# Autodesk Inventor assembly: Assembly5
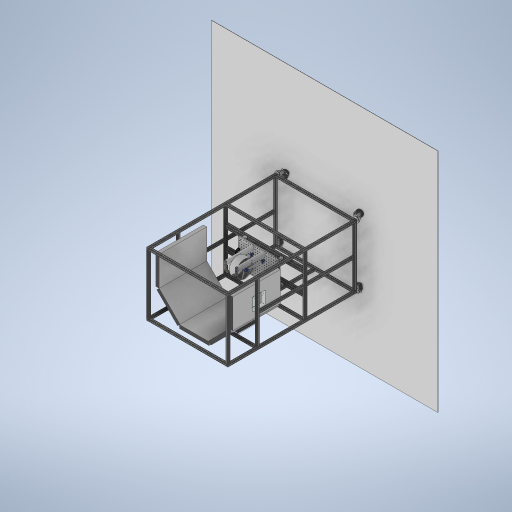
[picture p0: Inventor's stored thumbnail of the model, 512x512]
Saved by Autodesk Inventor 2024 (Build 280153000, 153)
## iProperties
Created: 2021-07-16
Part Number: Assembly5
Document SubType Name: Assembly
Designer: negre
Author: negre
## Documents named in this file (14)
- C:\Users\rosam\OneDrive\Documents\github_latest\Hardware\Tablet-Rig\Assemblies\Frame_training.iam
- C:\Users\rosam\OneDrive\Documents\github_latest\Hardware\Tablet-Rig\Parts\McMaster-Carr 47065T801\47065T801_T-Slotted Framing_57-inches.ipt
- C:\Users\rosam\OneDrive\Documents\github_latest\Hardware\Tablet-Rig\Parts\McMaster-Carr 47065T919\47065T919_T-Slotted Framing_caster.ipt
- C:\Users\rosam\OneDrive\Documents\github_latest\Hardware\Tablet-Rig\Assemblies\Wheel_w_board.iam
- C:\Users\rosam\OneDrive\Documents\github_latest\Hardware\Tablet-Rig\Parts\ThorLabs RS2\RS2-Step.ipt
- C:\Users\rosam\OneDrive\Documents\github_latest\Hardware\Tablet-Rig\Parts\McMaster-Carr 47065T801\47065T801_T-Slotted Framing_21-inches.ipt
- C:\Users\rosam\OneDrive\Documents\github_latest\Hardware\Tablet-Rig\Assemblies\Monitors_VESA-mountable.iam
- C:\Users\rosam\OneDrive\Documents\github_latest\Hardware\Tablet-Rig\Parts\Ground.ipt
- C:\Users\rosam\OneDrive\Documents\github_latest\Hardware\Tablet-Rig\Parts\McMaster-Carr 47065T801\47065T801_T-Slotted Framing_34-inches.ipt
- C:\Users\rosam\OneDrive\Documents\github_latest\Hardware\Tablet-Rig\Parts\McMaster-Carr 47065T803\47065T803_T-Slotted Framing_34-inches.ipt
- C:\Users\rosam\OneDrive\Documents\github_latest\Hardware\Tablet-Rig\Parts\McMaster-Carr 47065T801\47065T801_T-Slotted Framing_26-inches.ipt
- C:\Users\rosam\OneDrive\Documents\github_latest\Hardware\Tablet-Rig\Parts\McMaster-Carr 47065T801\47065T801_T-Slotted Framing_20-inches.ipt
- C:\Users\rosam\OneDrive\Documents\github_latest\Hardware\Tablet-Rig\Parts\VESA adapter bracket.ipt
- C:\Users\rosam\OneDrive\Documents\github_latest\Hardware\Tablet-Rig\Parts\McMaster-Carr 47065T801\47065T801_T-Slotted Framing_11-inches.ipt
## Components (46 placed, 13 different names)
1. 47065T801_T-Slotted Framing_57-inches:1 — Mate:1087, Mate:1088, Flush:895, Flush:1074, Flush:1075, Flush:1077, Flush:1079, Flush:1081, Mate:1282, Mate:1307, Flush:1144, Flush:1145, Mate:1309, Flush:1146, Flush:1155
2. 47065T801_T-Slotted Framing_57-inches:2 — Mate:1085, Mate:1086, Flush:1083, Flush:1084, Flush:1087, Mate:1281, Flush:1089, Mate:1305, Symmetry:1, Mate:1308, Mate:1311, Flush:1149, Mate:1313, Flush:1154, Flush:1193
3. 47065T801_T-Slotted Framing_57-inches:3 — Mate:1091, Mate:1092, Flush:895, Flush:1069, Mate:1275, Flush:1072, Flush:1073, Mate:1276, Flush:1076, Mate:1277, Flush:1078, Mate:1278, Flush:1080, Flush:1141, Flush:1142, Mate:1316, Flush:1160, Flush:1166, Flush:1167, Flush:1169
4. 47065T801_T-Slotted Framing_57-inches:4 — Mate:1089, Mate:1090, Mate:1279, Flush:1082, Flush:1085, Mate:1280, Flush:1086, Flush:1090, Flush:1141, Flush:1143, Symmetry:1, Mate:1321, Flush:1164, Flush:1165, Mate:1322, Flush:1168, Mate:1323, Mate:1327, Flush:1178, Mate:1330, Flush:1192
5. 47065T919_T-Slotted Framing_caster:1 — Mate:1087, Mate:1088
6. 47065T919_T-Slotted Framing_caster:2 — Mate:1091, Mate:1092
7. 47065T919_T-Slotted Framing_caster:3 — Mate:1089, Mate:1090
8. 47065T919_T-Slotted Framing_caster:4 — Mate:1085, Mate:1086, Mate:1274
9. Wheel_w_board:1 [sub-assembly] — Mate:1107, Mate:1108, Mate:1109, Mate:1110, Mate:1111, Mate:1112, Mate:1113, Mate:1114, Angle:1, Angle:2, Flush:1066, Flush:1067, Flush:1068, Flush:1136, Flush:1139
10. RS2-Step:1 — Mate:1107, Mate:1114, Mate:1302
11. RS2-Step:2 — Mate:1110, Mate:1111
12. RS2-Step:3 — Mate:1108, Mate:1113, Mate:1304
13. RS2-Step:4 — Mate:1109, Mate:1112
14. 47065T801_T-Slotted Framing_21-inches:1 — Mate:1310, Flush:1152, Mate:1312, Flush:1183, Flush:1184
15. 47065T801_T-Slotted Framing_21-inches:2 — Mate:1325, Flush:1176, Mate:1328, Flush:1182, Flush:1184
16. Monitors_VESA-mountable:1 [sub-assembly] — Angle:1, Angle:2, Flush:1066, Flush:1067, Flush:1068, Flush:1069, Angle:3, Angle:4, Flush:1071, Mate:1273, Mate:1318, Mate:1332, Flush:1186, Mate:1336, Flush:1190, Flush:1191, Flush:1194, Flush:1195, Flush:1196
17. Ground:1 — Mate:1270, Mate:1271, Flush:1070, Angle:3, Angle:4, Flush:1071, Mate:1273, Mate:1274, Angle:5, Mate:1306
18. 47065T801_T-Slotted Framing_34-inches:1 — Mate:1275, Flush:1072, Flush:1073, Flush:1074, Flush:1075, Mate:1282, Flush:1188, Flush:1189
19. 47065T801_T-Slotted Framing_34-inches:2 — Mate:1276, Flush:1076, Flush:1077, Flush:1147
20. 47065T801_T-Slotted Framing_34-inches:3 — Mate:1277, Flush:1078, Flush:1079, Flush:1091, Mate:1317, Flush:1162, Flush:1172
21. 47065T801_T-Slotted Framing_34-inches:4 — Mate:1278, Flush:1080, Flush:1081, Flush:1088, Flush:1140, Flush:1142, Flush:1151, Mate:1319, Flush:1163, Flush:1180
22. 47065T801_T-Slotted Framing_34-inches:5 — Mate:1279, Flush:1082, Flush:1083, Flush:1084, Flush:1085
23. 47065T801_T-Slotted Framing_34-inches:6 — Mate:1280, Flush:1086, Flush:1087, Flush:1088, Mate:1305, Flush:1140, Angle:5, Flush:1143, Flush:1150, Flush:1179
24. 47065T801_T-Slotted Framing_34-inches:7 — Mate:1281, Flush:1089, Flush:1090, Flush:1091, Flush:1148
25. 47065T803_T-Slotted Framing_34-inches:1 — Mate:1304, Flush:1139, Flush:1156, Flush:1174
26. 47065T803_T-Slotted Framing_34-inches:2 — Mate:1302, Flush:1136, Flush:1157, Mate:1324, Flush:1173, Mate:1326
27. 47065T801_T-Slotted Framing_26-inches:1 — Mate:1309, Flush:1146, Flush:1147, Flush:1148, Mate:1310, Flush:1152, Flush:1156, Flush:1157, Mate:1314, Flush:1158, Flush:1175, Mate:1326
28. 47065T801_T-Slotted Framing_26-inches:2 — Mate:1327, Flush:1178, Mate:1328, Flush:1179, Flush:1180
29. 47065T801_T-Slotted Framing_26-inches:3 — Mate:1323, Mate:1324, Flush:1172, Flush:1173, Flush:1174, Flush:1175, Mate:1325, Flush:1176, Mate:1329, Flush:1181
30. 47065T801_T-Slotted Framing_26-inches:4 — Mate:1322, Flush:1168, Flush:1169, Flush:1170, Flush:1171, Mate:1339
31. 47065T801_T-Slotted Framing_26-inches:5 — Mate:1307, Flush:1144, Flush:1145, Mate:1308, Flush:1185, Flush:1187
32. 47065T801_T-Slotted Framing_26-inches:6 — Mate:1311, Flush:1149, Flush:1150, Flush:1151, Mate:1312
33. 47065T801_T-Slotted Framing_26-inches:7 — Mate:1321, Flush:1164, Flush:1165, Flush:1166, Flush:1167
34. 47065T801_T-Slotted Framing_26-inches:8 — Mate:1313, Flush:1154, Flush:1155, Mate:1315, Flush:1161, Flush:1171, Mate:1331, Mate:1333
35. 47065T801_T-Slotted Framing_20-inches:1 — Mate:1314, Flush:1158, Mate:1315, Flush:1183
36. 47065T801_T-Slotted Framing_34-inches:8 — Mate:1316, Flush:1160, Flush:1161, Flush:1170, Mate:1335, Mate:1337
37. 47065T801_T-Slotted Framing_20-inches:2 — Mate:1317, Flush:1162, Mate:1318, Mate:1320
38. 47065T801_T-Slotted Framing_21-inches:3 — Mate:1319, Flush:1163, Mate:1320
39. 47065T801_T-Slotted Framing_20-inches:3 — Mate:1329, Flush:1181, Flush:1182, Mate:1330
40. VESA adapter bracket:1 — Mate:1338, Flush:1190, Flush:1194
41. VESA adapter bracket:2 — Mate:1331, Flush:1185, Flush:1193
42. VESA adapter bracket:3 — Mate:1339, Flush:1191, Flush:1192
43. VESA adapter bracket:4 — Mate:1334, Flush:1187, Flush:1196
44. VESA adapter bracket:5 — Mate:1335, Flush:1188, Flush:1195
45. 47065T801_T-Slotted Framing_11-inches:1 — Mate:1336, Flush:1189, Mate:1337, Mate:1338
46. 47065T801_T-Slotted Framing_11-inches:2 — Mate:1332, Mate:1333, Flush:1186, Mate:1334
## Relationships (154: Flush 83, Mate 65, Angle 5, Symmetry 1)
- Mate:1085: 47065T801_T-Slotted Framing_57-inches:2 ↔ 47065T919_T-Slotted Framing_caster:4
- Mate:1086: 47065T801_T-Slotted Framing_57-inches:2 ↔ 47065T919_T-Slotted Framing_caster:4
- Mate:1087: 47065T801_T-Slotted Framing_57-inches:1 ↔ 47065T919_T-Slotted Framing_caster:1
- Mate:1088: 47065T801_T-Slotted Framing_57-inches:1 ↔ 47065T919_T-Slotted Framing_caster:1
- Mate:1089: 47065T801_T-Slotted Framing_57-inches:4 ↔ 47065T919_T-Slotted Framing_caster:3
- Mate:1090: 47065T801_T-Slotted Framing_57-inches:4 ↔ 47065T919_T-Slotted Framing_caster:3
- Mate:1091: 47065T801_T-Slotted Framing_57-inches:3 ↔ 47065T919_T-Slotted Framing_caster:2
- Mate:1092: 47065T801_T-Slotted Framing_57-inches:3 ↔ 47065T919_T-Slotted Framing_caster:2
- Flush:895: 47065T801_T-Slotted Framing_57-inches:1 ↔ 47065T801_T-Slotted Framing_57-inches:3
- Mate:1107: Wheel_w_board:1 ↔ RS2-Step:1
- Mate:1108: Wheel_w_board:1 ↔ RS2-Step:3
- Mate:1109: Wheel_w_board:1 ↔ RS2-Step:4
- Mate:1110: Wheel_w_board:1 ↔ RS2-Step:2
- Mate:1111: Wheel_w_board:1 ↔ RS2-Step:2
- Mate:1112: Wheel_w_board:1 ↔ RS2-Step:4
- Mate:1113: Wheel_w_board:1 ↔ RS2-Step:3
- Mate:1114: Wheel_w_board:1 ↔ RS2-Step:1
- Angle:1 (0 deg): Wheel_w_board:1 ↔ Monitors_VESA-mountable:1
- Angle:2 (180 deg): Wheel_w_board:1 ↔ Monitors_VESA-mountable:1
- Flush:1066: Wheel_w_board:1 ↔ Monitors_VESA-mountable:1
- Flush:1067 (381 mm): Wheel_w_board:1 ↔ Monitors_VESA-mountable:1
- Flush:1068 (-127 mm): Wheel_w_board:1 ↔ Monitors_VESA-mountable:1
- Flush:1069 (-25.4 mm): 47065T801_T-Slotted Framing_57-inches:3 ↔ Monitors_VESA-mountable:1
- Mate:1270: Ground:1
- Mate:1271: Ground:1
- Flush:1070: Ground:1
- Angle:3 (0 deg): Monitors_VESA-mountable:1 ↔ Ground:1
- Angle:4 (0 deg): Monitors_VESA-mountable:1 ↔ Ground:1
- Flush:1071: Monitors_VESA-mountable:1 ↔ Ground:1
- Mate:1273: Monitors_VESA-mountable:1 ↔ Ground:1
- Mate:1274 (38.1 mm): 47065T919_T-Slotted Framing_caster:4 ↔ Ground:1
- Mate:1275: 47065T801_T-Slotted Framing_57-inches:3 ↔ 47065T801_T-Slotted Framing_34-inches:1
- Flush:1072: 47065T801_T-Slotted Framing_57-inches:3 ↔ 47065T801_T-Slotted Framing_34-inches:1
- Flush:1073: 47065T801_T-Slotted Framing_57-inches:3 ↔ 47065T801_T-Slotted Framing_34-inches:1
- Flush:1074: 47065T801_T-Slotted Framing_57-inches:1 ↔ 47065T801_T-Slotted Framing_34-inches:1
- Flush:1075: 47065T801_T-Slotted Framing_57-inches:1 ↔ 47065T801_T-Slotted Framing_34-inches:1
- Mate:1276: 47065T801_T-Slotted Framing_57-inches:3 ↔ 47065T801_T-Slotted Framing_34-inches:2
- Flush:1076: 47065T801_T-Slotted Framing_57-inches:3 ↔ 47065T801_T-Slotted Framing_34-inches:2
- Flush:1077: 47065T801_T-Slotted Framing_57-inches:1 ↔ 47065T801_T-Slotted Framing_34-inches:2
- Mate:1277: 47065T801_T-Slotted Framing_57-inches:3 ↔ 47065T801_T-Slotted Framing_34-inches:3
- Flush:1078: 47065T801_T-Slotted Framing_57-inches:3 ↔ 47065T801_T-Slotted Framing_34-inches:3
- Flush:1079: 47065T801_T-Slotted Framing_57-inches:1 ↔ 47065T801_T-Slotted Framing_34-inches:3
- Mate:1278: 47065T801_T-Slotted Framing_57-inches:3 ↔ 47065T801_T-Slotted Framing_34-inches:4
- Flush:1080: 47065T801_T-Slotted Framing_57-inches:3 ↔ 47065T801_T-Slotted Framing_34-inches:4
- Flush:1081: 47065T801_T-Slotted Framing_57-inches:1 ↔ 47065T801_T-Slotted Framing_34-inches:4
- Mate:1279: 47065T801_T-Slotted Framing_57-inches:4 ↔ 47065T801_T-Slotted Framing_34-inches:5
- Flush:1082: 47065T801_T-Slotted Framing_57-inches:4 ↔ 47065T801_T-Slotted Framing_34-inches:5
- Flush:1083: 47065T801_T-Slotted Framing_57-inches:2 ↔ 47065T801_T-Slotted Framing_34-inches:5
- Flush:1084: 47065T801_T-Slotted Framing_57-inches:2 ↔ 47065T801_T-Slotted Framing_34-inches:5
- Flush:1085: 47065T801_T-Slotted Framing_57-inches:4 ↔ 47065T801_T-Slotted Framing_34-inches:5
- Mate:1280: 47065T801_T-Slotted Framing_57-inches:4 ↔ 47065T801_T-Slotted Framing_34-inches:6
- Flush:1086: 47065T801_T-Slotted Framing_57-inches:4 ↔ 47065T801_T-Slotted Framing_34-inches:6
- Flush:1087: 47065T801_T-Slotted Framing_57-inches:2 ↔ 47065T801_T-Slotted Framing_34-inches:6
- Flush:1088: 47065T801_T-Slotted Framing_34-inches:4 ↔ 47065T801_T-Slotted Framing_34-inches:6
- Mate:1281: 47065T801_T-Slotted Framing_57-inches:2 ↔ 47065T801_T-Slotted Framing_34-inches:7
- Flush:1089: 47065T801_T-Slotted Framing_57-inches:2 ↔ 47065T801_T-Slotted Framing_34-inches:7
- Flush:1090: 47065T801_T-Slotted Framing_57-inches:4 ↔ 47065T801_T-Slotted Framing_34-inches:7
- Flush:1091: 47065T801_T-Slotted Framing_34-inches:3 ↔ 47065T801_T-Slotted Framing_34-inches:7
- Mate:1282: 47065T801_T-Slotted Framing_57-inches:1 ↔ 47065T801_T-Slotted Framing_34-inches:1
- Mate:1302: RS2-Step:1 ↔ 47065T803_T-Slotted Framing_34-inches:2
- Flush:1136 (12.7 mm): Wheel_w_board:1 ↔ 47065T803_T-Slotted Framing_34-inches:2
- Mate:1304: RS2-Step:3 ↔ 47065T803_T-Slotted Framing_34-inches:1
- Flush:1139 (12.7 mm): Wheel_w_board:1 ↔ 47065T803_T-Slotted Framing_34-inches:1
- Mate:1305: 47065T801_T-Slotted Framing_57-inches:2 ↔ 47065T801_T-Slotted Framing_34-inches:6
- Flush:1140: 47065T801_T-Slotted Framing_34-inches:4 ↔ 47065T801_T-Slotted Framing_34-inches:6
- Flush:1141: 47065T801_T-Slotted Framing_57-inches:3 ↔ 47065T801_T-Slotted Framing_57-inches:4
- Angle:5 (0 deg): Ground:1 ↔ 47065T801_T-Slotted Framing_34-inches:6
- Flush:1142: 47065T801_T-Slotted Framing_57-inches:3 ↔ 47065T801_T-Slotted Framing_34-inches:4
- Flush:1143: 47065T801_T-Slotted Framing_57-inches:4 ↔ 47065T801_T-Slotted Framing_34-inches:6
- Symmetry:1: 47065T801_T-Slotted Framing_57-inches:2 ↔ 47065T801_T-Slotted Framing_57-inches:4
- Mate:1306: Ground:1
- Mate:1307: 47065T801_T-Slotted Framing_57-inches:1 ↔ 47065T801_T-Slotted Framing_26-inches:5
- Flush:1144: 47065T801_T-Slotted Framing_57-inches:1 ↔ 47065T801_T-Slotted Framing_26-inches:5
- Flush:1145: 47065T801_T-Slotted Framing_57-inches:1 ↔ 47065T801_T-Slotted Framing_26-inches:5
- Mate:1308: 47065T801_T-Slotted Framing_57-inches:2 ↔ 47065T801_T-Slotted Framing_26-inches:5
- Mate:1309: 47065T801_T-Slotted Framing_57-inches:1 ↔ 47065T801_T-Slotted Framing_26-inches:1
- Flush:1146: 47065T801_T-Slotted Framing_57-inches:1 ↔ 47065T801_T-Slotted Framing_26-inches:1
- Flush:1147: 47065T801_T-Slotted Framing_34-inches:2 ↔ 47065T801_T-Slotted Framing_26-inches:1
- Flush:1148: 47065T801_T-Slotted Framing_34-inches:7 ↔ 47065T801_T-Slotted Framing_26-inches:1
- Mate:1310: 47065T801_T-Slotted Framing_21-inches:1 ↔ 47065T801_T-Slotted Framing_26-inches:1
- Mate:1311: 47065T801_T-Slotted Framing_57-inches:2 ↔ 47065T801_T-Slotted Framing_26-inches:6
- Flush:1149: 47065T801_T-Slotted Framing_57-inches:2 ↔ 47065T801_T-Slotted Framing_26-inches:6
- Flush:1150: 47065T801_T-Slotted Framing_34-inches:6 ↔ 47065T801_T-Slotted Framing_26-inches:6
- Flush:1151: 47065T801_T-Slotted Framing_34-inches:4 ↔ 47065T801_T-Slotted Framing_26-inches:6
- Flush:1152: 47065T801_T-Slotted Framing_21-inches:1 ↔ 47065T801_T-Slotted Framing_26-inches:1
- Mate:1312: 47065T801_T-Slotted Framing_21-inches:1 ↔ 47065T801_T-Slotted Framing_26-inches:6
- Mate:1313: 47065T801_T-Slotted Framing_57-inches:2 ↔ 47065T801_T-Slotted Framing_26-inches:8
- Flush:1154: 47065T801_T-Slotted Framing_57-inches:2 ↔ 47065T801_T-Slotted Framing_26-inches:8
- Flush:1155: 47065T801_T-Slotted Framing_57-inches:1 ↔ 47065T801_T-Slotted Framing_26-inches:8
- Flush:1156: 47065T803_T-Slotted Framing_34-inches:1 ↔ 47065T801_T-Slotted Framing_26-inches:1
- Flush:1157: 47065T803_T-Slotted Framing_34-inches:2 ↔ 47065T801_T-Slotted Framing_26-inches:1
- Mate:1314: 47065T801_T-Slotted Framing_26-inches:1 ↔ 47065T801_T-Slotted Framing_20-inches:1
- Flush:1158: 47065T801_T-Slotted Framing_26-inches:1 ↔ 47065T801_T-Slotted Framing_20-inches:1
- Mate:1315: 47065T801_T-Slotted Framing_26-inches:8 ↔ 47065T801_T-Slotted Framing_20-inches:1
- Mate:1316: 47065T801_T-Slotted Framing_57-inches:3 ↔ 47065T801_T-Slotted Framing_34-inches:8
- Flush:1160: 47065T801_T-Slotted Framing_57-inches:3 ↔ 47065T801_T-Slotted Framing_34-inches:8
- Flush:1161: 47065T801_T-Slotted Framing_26-inches:8 ↔ 47065T801_T-Slotted Framing_34-inches:8
- Mate:1317: 47065T801_T-Slotted Framing_34-inches:3 ↔ 47065T801_T-Slotted Framing_20-inches:2
- Flush:1162: 47065T801_T-Slotted Framing_34-inches:3 ↔ 47065T801_T-Slotted Framing_20-inches:2
- Mate:1318: Monitors_VESA-mountable:1 ↔ 47065T801_T-Slotted Framing_20-inches:2
- Mate:1319: 47065T801_T-Slotted Framing_34-inches:4 ↔ 47065T801_T-Slotted Framing_21-inches:3
- Flush:1163: 47065T801_T-Slotted Framing_34-inches:4 ↔ 47065T801_T-Slotted Framing_21-inches:3
- Mate:1320: 47065T801_T-Slotted Framing_20-inches:2 ↔ 47065T801_T-Slotted Framing_21-inches:3
- Mate:1321: 47065T801_T-Slotted Framing_57-inches:4 ↔ 47065T801_T-Slotted Framing_26-inches:7
- Flush:1164: 47065T801_T-Slotted Framing_57-inches:4 ↔ 47065T801_T-Slotted Framing_26-inches:7
- Flush:1165: 47065T801_T-Slotted Framing_57-inches:4 ↔ 47065T801_T-Slotted Framing_26-inches:7
- Flush:1166: 47065T801_T-Slotted Framing_57-inches:3 ↔ 47065T801_T-Slotted Framing_26-inches:7
- Flush:1167: 47065T801_T-Slotted Framing_57-inches:3 ↔ 47065T801_T-Slotted Framing_26-inches:7
- Mate:1322: 47065T801_T-Slotted Framing_57-inches:4 ↔ 47065T801_T-Slotted Framing_26-inches:4
- Flush:1168: 47065T801_T-Slotted Framing_57-inches:4 ↔ 47065T801_T-Slotted Framing_26-inches:4
- Flush:1169: 47065T801_T-Slotted Framing_57-inches:3 ↔ 47065T801_T-Slotted Framing_26-inches:4
- Flush:1170: 47065T801_T-Slotted Framing_26-inches:4 ↔ 47065T801_T-Slotted Framing_34-inches:8
- Flush:1171: 47065T801_T-Slotted Framing_26-inches:4 ↔ 47065T801_T-Slotted Framing_26-inches:8
- Mate:1323: 47065T801_T-Slotted Framing_57-inches:4 ↔ 47065T801_T-Slotted Framing_26-inches:3
- Mate:1324: 47065T803_T-Slotted Framing_34-inches:2 ↔ 47065T801_T-Slotted Framing_26-inches:3
- Flush:1172: 47065T801_T-Slotted Framing_34-inches:3 ↔ 47065T801_T-Slotted Framing_26-inches:3
- Flush:1173: 47065T803_T-Slotted Framing_34-inches:2 ↔ 47065T801_T-Slotted Framing_26-inches:3
- Flush:1174: 47065T803_T-Slotted Framing_34-inches:1 ↔ 47065T801_T-Slotted Framing_26-inches:3
- Flush:1175: 47065T801_T-Slotted Framing_26-inches:1 ↔ 47065T801_T-Slotted Framing_26-inches:3
- Mate:1325: 47065T801_T-Slotted Framing_21-inches:2 ↔ 47065T801_T-Slotted Framing_26-inches:3
- Flush:1176: 47065T801_T-Slotted Framing_21-inches:2 ↔ 47065T801_T-Slotted Framing_26-inches:3
- Mate:1326: 47065T803_T-Slotted Framing_34-inches:2 ↔ 47065T801_T-Slotted Framing_26-inches:1
- Mate:1327: 47065T801_T-Slotted Framing_57-inches:4 ↔ 47065T801_T-Slotted Framing_26-inches:2
- Flush:1178: 47065T801_T-Slotted Framing_57-inches:4 ↔ 47065T801_T-Slotted Framing_26-inches:2
- Mate:1328: 47065T801_T-Slotted Framing_21-inches:2 ↔ 47065T801_T-Slotted Framing_26-inches:2
- Flush:1179: 47065T801_T-Slotted Framing_34-inches:6 ↔ 47065T801_T-Slotted Framing_26-inches:2
- Flush:1180: 47065T801_T-Slotted Framing_34-inches:4 ↔ 47065T801_T-Slotted Framing_26-inches:2
- Mate:1329: 47065T801_T-Slotted Framing_26-inches:3 ↔ 47065T801_T-Slotted Framing_20-inches:3
- Flush:1181: 47065T801_T-Slotted Framing_26-inches:3 ↔ 47065T801_T-Slotted Framing_20-inches:3
- Flush:1182: 47065T801_T-Slotted Framing_21-inches:2 ↔ 47065T801_T-Slotted Framing_20-inches:3
- Flush:1183: 47065T801_T-Slotted Framing_21-inches:1 ↔ 47065T801_T-Slotted Framing_20-inches:1
- Flush:1184: 47065T801_T-Slotted Framing_21-inches:1 ↔ 47065T801_T-Slotted Framing_21-inches:2
- Mate:1330 (317.5 mm): 47065T801_T-Slotted Framing_57-inches:4 ↔ 47065T801_T-Slotted Framing_20-inches:3
- Mate:1331: 47065T801_T-Slotted Framing_26-inches:8 ↔ VESA adapter bracket:2
- Flush:1185 (273.05 mm): 47065T801_T-Slotted Framing_26-inches:5 ↔ VESA adapter bracket:2
- Mate:1332: Monitors_VESA-mountable:1 ↔ 47065T801_T-Slotted Framing_11-inches:2
- Mate:1333 (12.7 mm): 47065T801_T-Slotted Framing_26-inches:8 ↔ 47065T801_T-Slotted Framing_11-inches:2
- Flush:1186 (254 mm): Monitors_VESA-mountable:1 ↔ 47065T801_T-Slotted Framing_11-inches:2
- Mate:1334: VESA adapter bracket:4 ↔ 47065T801_T-Slotted Framing_11-inches:2
- Flush:1187 (266.7 mm): 47065T801_T-Slotted Framing_26-inches:5 ↔ VESA adapter bracket:4
- Mate:1335: 47065T801_T-Slotted Framing_34-inches:8 ↔ VESA adapter bracket:5
- Flush:1188 (266.7 mm): 47065T801_T-Slotted Framing_34-inches:1 ↔ VESA adapter bracket:5
- Mate:1336: Monitors_VESA-mountable:1 ↔ 47065T801_T-Slotted Framing_11-inches:1
- Flush:1189 (330.2 mm): 47065T801_T-Slotted Framing_34-inches:1 ↔ 47065T801_T-Slotted Framing_11-inches:1
- Mate:1337 (12.7 mm): 47065T801_T-Slotted Framing_34-inches:8 ↔ 47065T801_T-Slotted Framing_11-inches:1
- Mate:1338: VESA adapter bracket:1 ↔ 47065T801_T-Slotted Framing_11-inches:1
- Flush:1190 (190.5 mm): Monitors_VESA-mountable:1 ↔ VESA adapter bracket:1
- Mate:1339: 47065T801_T-Slotted Framing_26-inches:4 ↔ VESA adapter bracket:3
- Flush:1191 (190.5 mm): Monitors_VESA-mountable:1 ↔ VESA adapter bracket:3
- Flush:1192 (177.8 mm): 47065T801_T-Slotted Framing_57-inches:4 ↔ VESA adapter bracket:3
- Flush:1193 (165.1 mm): 47065T801_T-Slotted Framing_57-inches:2 ↔ VESA adapter bracket:2
- Flush:1194 (88.9 mm): Monitors_VESA-mountable:1 ↔ VESA adapter bracket:1
- Flush:1195 (88.9 mm): Monitors_VESA-mountable:1 ↔ VESA adapter bracket:5
- Flush:1196 (88.9 mm): Monitors_VESA-mountable:1 ↔ VESA adapter bracket:4
